# Autodesk Inventor assembly: HB8_910.1-sunhub8_pcb
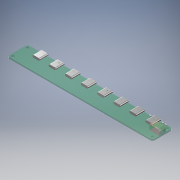
[picture p0: Inventor's stored thumbnail of the model, 180x180]
Saved by Autodesk Inventor 2019 (Build 230136000, 136)
## iProperties
Created: 2019-03-01
Part Number: HB8_910.1-sunhub8_pcb
Document SubType Name: Assembly
Designer: Rene
Author: Rene
## Documents named in this file (5)
- C:\dev\c-scape\hardponics\dwg\sunhub\HB8_910.1-sunhub8_pcb.iam
- C:\dev\c-scape\hardponics\dwg\sunhub\SH8_003.1-sunhub8-PCB.ipt
- C:\dev\c-scape\hardponics\dwg\sunhub\XGEN_USB-C_socket_pcb.ipt
- C:\dev\c-scape\hardponics\dwg\sunhub\XGEN_LED-sidelooker_green.ipt
- C:\dev\c-scape\hardponics\dwg\sunhub\XGEN_LED-sidelooker_red.ipt
## Components (12 placed, 4 different names)
1. SH8_003.1-sunhub8-PCB:1 — Mate:1, Flush:1, Mate:2, Flush:2, Mate:3, Flush:3
2. XGEN_LED-sidelooker_red:1 — Mate:3, Flush:3
3. XGEN_USB-C_socket_pcb:1 — Mate:1, Flush:1
4. XGEN_USB-C_socket_pcb:2
5. XGEN_USB-C_socket_pcb:3
6. XGEN_USB-C_socket_pcb:4
7. XGEN_USB-C_socket_pcb:5
8. XGEN_USB-C_socket_pcb:6
9. XGEN_USB-C_socket_pcb:7
10. XGEN_USB-C_socket_pcb:8
11. XGEN_LED-sidelooker_green:1 — Mate:2, Flush:2
12. XGEN_LED-sidelooker_green:2
## Component patterns: (8 elements, first: XGEN_USB-C_socket_pcb:1), (2 elements, first: XGEN_LED-sidelooker_green:1)
## Relationships (6: Mate 3, Flush 3)
- Mate:1: SH8_003.1-sunhub8-PCB:1 ↔ XGEN_USB-C_socket_pcb:1
- Flush:1: SH8_003.1-sunhub8-PCB:1 ↔ XGEN_USB-C_socket_pcb:1
- Mate:2: SH8_003.1-sunhub8-PCB:1 ↔ XGEN_LED-sidelooker_green:1
- Flush:2: SH8_003.1-sunhub8-PCB:1 ↔ XGEN_LED-sidelooker_green:1
- Mate:3: SH8_003.1-sunhub8-PCB:1 ↔ XGEN_LED-sidelooker_red:1
- Flush:3: SH8_003.1-sunhub8-PCB:1 ↔ XGEN_LED-sidelooker_red:1
